# Autodesk Inventor assembly: robot_frame_layer2
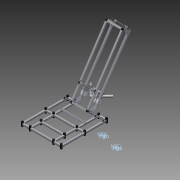
[picture p0: Inventor's stored thumbnail of the model, 180x180]
Saved by Autodesk Inventor 2011 (Build 150239000, 239)
## iProperties
Created: 2013-01-17
Part Number: robot_frame_layer2
Document SubType Name: Assembly
Designer: Christopher
Author: Christopher
## Documents named in this file (19)
- F:\Users\Christopher\Documents\GitHub\2013CAD\2013 robot\forklift\robot parts\robot_frame_layer2.iam
- F:\Users\Christopher\Documents\GitHub\2013CAD\2013 robot\forklift\robot parts\1tube_4_layer1_outside.ipt
- F:\Users\Christopher\Documents\GitHub\2013CAD\2013 robot\forklift\robot parts\1tube_6_layer1_boardsupportsupport.ipt
- F:\Users\Christopher\Documents\GitHub\2013CAD\2013 robot\forklift\robot parts\1tube_6_layer1_motorsupport.ipt
- F:\Users\Christopher\Documents\GitHub\2013CAD\2013 robot\forklift\robot parts\1tube_14_layer1_innersupport.ipt
- F:\Users\Christopher\Documents\GitHub\2013CAD\2013 robot\forklift\robot parts\1tube_14_layer1_inside.ipt
- F:\Users\Christopher\Documents\GitHub\2013CAD\2013 robot\forklift\robot parts\1tube_14_layer1_outside.ipt
- F:\Users\Christopher\Documents\GitHub\2013CAD\2013 robot\forklift\Misc parts\4-way corner.ipt
- F:\Users\Christopher\Documents\GitHub\2013CAD\2013 robot\forklift\Misc parts\5-way corner.ipt
- F:\Users\Christopher\Documents\GitHub\2013CAD\2013 robot\forklift\Misc parts\.5inch_side_bearing.ipt
- F:\Users\Christopher\Documents\GitHub\2013CAD\2013 robot\forklift\Misc parts\1.5_bolt_.25_20.ipt
- F:\Users\Christopher\Documents\GitHub\2013CAD\2013 robot\forklift\Misc parts\nut_.25_20.ipt
- F:\Users\Christopher\Documents\GitHub\2013CAD\2013 robot\forklift\Misc parts\.5_inch_axle_bushing.ipt
- F:\Users\Christopher\Documents\GitHub\2013CAD\2013 robot\forklift\robot parts\1tube_13_layer2_side.ipt
- F:\Users\Christopher\Documents\GitHub\2013CAD\2013 robot\forklift\Misc parts\6-way corner.ipt
- F:\Users\Christopher\Documents\GitHub\2013CAD\2013 robot\forklift\frame parts\0.5unkeyedaxle_26.ipt
- F:\Users\Christopher\Documents\GitHub\2013CAD\2013 robot\forklift\frame parts\forklift_1_0.iam
- F:\Users\Christopher\Documents\GitHub\2013CAD\2013 robot\forklift\Misc parts\steel_p60_mounting _plate.ipt
- F:\Users\Christopher\Documents\GitHub\2013CAD\2013 robot\forklift\Misc parts\hack_p60.ipt
## Components (66 placed, 18 different names)
1. 1tube_4_layer1_outside:1 — Mate:231, Mate:232, Mate:233, Mate:237, Mate:238, Mate:239
2. 1tube_6_layer1_boardsupportsupport:1 — Mate:225, Mate:226, Mate:227
3. 1tube_6_layer1_motorsupport:1 — Mate:221, Mate:222, Mate:223
4. 1tube_14_layer1_innersupport:1 — Mate:182, Mate:186, Mate:195, Mate:218, Mate:219, Mate:224
5. 1tube_14_layer1_outside:1 — Mate:234, Mate:235, Mate:236
6. 1tube_4_layer1_outside:2 — Mate:204, Flush:20, Mate:205, Mate:206, Mate:207, Mate:208
7. 1tube_14_layer1_innersupport:2 — Mate:175, Mate:176, Mate:185, Mate:192, Mate:193, Mate:194
8. 1tube_6_layer1_motorsupport:2 — Mate:173, Mate:177, Mate:179, Mate:183, Flush:17, Mate:184
9. 1tube_6_layer1_boardsupportsupport:2 — Mate:187, Mate:188, Mate:189, Mate:190, Mate:191
10. 1tube_4_layer1_outside:3 — Mate:164, Mate:165, Mate:166, Flush:18
11. 1tube_4_layer1_outside:4 — Mate:149, Mate:150, Mate:151, Mate:155, Mate:156, Flush:12
12. 1tube_4_layer1_outside:5 — Mate:159, Mate:160, Mate:161, Mate:178, Mate:241
13. 1tube_4_layer1_outside:6 — Mate:196, Mate:197, Mate:198, Mate:199, Mate:200, Mate:201, Mate:202
14. 1tube_14_layer1_inside:2 — Mate:162, Mate:167, Flush:16, Mate:168, Mate:169, Mate:170, Mate:171
15. 1tube_14_layer1_inside:3 — Flush:19, Mate:203, Mate:220, Mate:228, Mate:229, Mate:230
16. .5inch_side_bearing:1 — Insert:5, Insert:6, Insert:18, Insert:41, Insert:42, Insert:59
17. .5inch_side_bearing:2 — Insert:7, Insert:8, Insert:19, Insert:36, Insert:45, Insert:46
18. 1.5_bolt_.25_20:1 — Insert:6
19. 1.5_bolt_.25_20:2 — Insert:5
20. 1.5_bolt_.25_20:3 — Insert:7
21. 1.5_bolt_.25_20:4 — Insert:8
22. .5_inch_axle_bushing:1 — Insert:18
23. .5_inch_axle_bushing:2 — Insert:19
24. .5_inch_axle_bushing:6 — Insert:57, Insert:58, Insert:59
25. .5inch_side_bearing:3 — Insert:27, Insert:28, Insert:37, Insert:39, Insert:43, Insert:44
26. .5inch_side_bearing:4 — Insert:29, Insert:30, Insert:38, Insert:40, Insert:47, Insert:48
27. 1.5_bolt_.25_20:5 — Insert:28
28. 1.5_bolt_.25_20:6 — Insert:30
29. 1.5_bolt_.25_20:7 — Insert:29
30. 1.5_bolt_.25_20:8 — Insert:27
31. nut_.25_20:8 — Insert:56
32. .5_inch_axle_bushing:7 — Insert:36
33. .5_inch_axle_bushing:8 — Insert:37
34. .5_inch_axle_bushing:9 — Insert:38
35. .5_inch_axle_bushing:10 — Insert:39
36. .5_inch_axle_bushing:11 — Insert:40
37. 5-way corner:3 — Mate:218, Mate:219, Mate:224, Mate:225, Mate:226, Mate:227
38. 4-way corner:10 — Mate:155, Mate:156, Flush:12, Mate:157, Mate:158, Flush:13
39. 4-way corner:11 — Mate:149, Mate:150, Mate:151, Mate:152, Mate:153, Mate:154
40. 1tube_13_layer2_side:1 — Mate:157, Mate:158, Flush:13, Mate:172, Mate:174, Insert:43, Insert:44, Insert:49, Insert:50, Mate:240, Flush:21
41. 1tube_13_layer2_side:2 — Mate:152, Mate:153, Mate:154, Mate:163, Flush:14, Flush:15, Insert:41, Insert:42, Insert:51, Insert:52
42. 1tube_13_layer2_side:3 — Mate:212, Mate:213, Mate:214, Insert:47, Insert:48, Insert:55, Insert:56
43. 1tube_13_layer2_side:4 — Mate:209, Mate:210, Mate:211, Mate:215, Mate:216, Mate:217, Insert:45, Insert:46, Insert:53, Insert:54
44. 5-way corner:4 — Mate:159, Mate:160, Mate:161, Mate:162, Mate:163, Flush:14, Flush:15, Mate:168, Mate:169, Mate:170
45. 4-way corner:12 — Mate:164, Mate:165, Mate:166, Mate:167, Flush:16, Mate:171
46. 6-way corner:1 — Mate:172, Mate:173, Mate:174, Mate:175, Mate:176, Mate:177, Mate:178, Mate:179, Mate:185
47. 5-way corner:5 — Mate:182, Mate:183, Flush:17, Mate:184, Mate:186, Mate:187, Mate:188, Mate:189, Mate:195
48. 5-way corner:6 — Mate:190, Mate:191, Flush:18, Mate:234, Mate:235, Mate:236
49. 6-way corner:2 — Mate:192, Mate:193, Mate:194, Mate:196, Mate:197, Mate:198, Mate:215, Mate:216, Mate:217, Mate:221, Mate:222, Mate:223
50. 5-way corner:7 — Mate:199, Flush:19, Mate:200, Mate:201, Mate:202, Mate:203, Mate:220
51. 4-way corner:13 — Mate:204, Flush:20, Mate:205, Mate:209, Mate:210, Mate:211
52. 4-way corner:14 — Mate:206, Mate:207, Mate:208, Mate:212, Mate:213, Mate:214
53. 4-way corner:15 — Mate:228, Mate:229, Mate:230, Mate:231, Mate:232, Mate:233
54. 5-way corner:8 — Mate:237, Mate:238, Mate:239
55. nut_.25_20:9 — Insert:49
56. nut_.25_20:10 — Insert:50
57. nut_.25_20:11 — Insert:51
58. nut_.25_20:12 — Insert:52
59. nut_.25_20:13 — Insert:53
60. nut_.25_20:14 — Insert:55
61. nut_.25_20:15 — Insert:54
62. 0.5unkeyedaxle_26:1 — Insert:57
63. forklift_1_0:1 [sub-assembly] — Insert:58
64. steel_p60_mounting _plate:1 — Mate:240, Flush:21, Mate:241, Mate:242, Flush:22, Flush:23, Mate:243, Flush:24, Flush:25
65. hack_p60:1 — Mate:242, Flush:22, Flush:23
66. hack_p60:2 — Mate:243, Flush:24, Flush:25
## Relationships (141: Mate 93, Insert 34, Flush 14)
- Insert:5: .5inch_side_bearing:1 ↔ 1.5_bolt_.25_20:2
- Insert:6: .5inch_side_bearing:1 ↔ 1.5_bolt_.25_20:1
- Insert:7: .5inch_side_bearing:2 ↔ 1.5_bolt_.25_20:3
- Insert:8: .5inch_side_bearing:2 ↔ 1.5_bolt_.25_20:4
- Insert:18: .5inch_side_bearing:1 ↔ .5_inch_axle_bushing:1
- Insert:19: .5inch_side_bearing:2 ↔ .5_inch_axle_bushing:2
- Insert:27: .5inch_side_bearing:3 ↔ 1.5_bolt_.25_20:8
- Insert:28: .5inch_side_bearing:3 ↔ 1.5_bolt_.25_20:5
- Insert:29: .5inch_side_bearing:4 ↔ 1.5_bolt_.25_20:7
- Insert:30: .5inch_side_bearing:4 ↔ 1.5_bolt_.25_20:6
- Insert:36: .5inch_side_bearing:2 ↔ .5_inch_axle_bushing:7
- Insert:37: .5inch_side_bearing:3 ↔ .5_inch_axle_bushing:8
- Insert:38: .5inch_side_bearing:4 ↔ .5_inch_axle_bushing:9
- Insert:39: .5inch_side_bearing:3 ↔ .5_inch_axle_bushing:10
- Insert:40: .5inch_side_bearing:4 ↔ .5_inch_axle_bushing:11
- Mate:149: 1tube_4_layer1_outside:4 ↔ 4-way corner:11
- Mate:150: 1tube_4_layer1_outside:4 ↔ 4-way corner:11
- Mate:151: 1tube_4_layer1_outside:4 ↔ 4-way corner:11
- Mate:152: 4-way corner:11 ↔ 1tube_13_layer2_side:2
- Mate:153: 4-way corner:11 ↔ 1tube_13_layer2_side:2
- Mate:154: 4-way corner:11 ↔ 1tube_13_layer2_side:2
- Mate:155: 1tube_4_layer1_outside:4 ↔ 4-way corner:10
- Mate:156: 1tube_4_layer1_outside:4 ↔ 4-way corner:10
- Flush:12: 1tube_4_layer1_outside:4 ↔ 4-way corner:10
- Mate:157: 4-way corner:10 ↔ 1tube_13_layer2_side:1
- Mate:158: 4-way corner:10 ↔ 1tube_13_layer2_side:1
- Flush:13: 4-way corner:10 ↔ 1tube_13_layer2_side:1
- Mate:159: 1tube_4_layer1_outside:5 ↔ 5-way corner:4
- Mate:160: 1tube_4_layer1_outside:5 ↔ 5-way corner:4
- Mate:161: 1tube_4_layer1_outside:5 ↔ 5-way corner:4
- Mate:162: 1tube_14_layer1_inside:2 ↔ 5-way corner:4
- Mate:163: 1tube_13_layer2_side:2 ↔ 5-way corner:4
- Flush:14: 1tube_13_layer2_side:2 ↔ 5-way corner:4
- Flush:15: 1tube_13_layer2_side:2 ↔ 5-way corner:4
- Mate:164: 1tube_4_layer1_outside:3 ↔ 4-way corner:12
- Mate:165: 1tube_4_layer1_outside:3 ↔ 4-way corner:12
- Mate:166: 1tube_4_layer1_outside:3 ↔ 4-way corner:12
- Mate:167: 1tube_14_layer1_inside:2 ↔ 4-way corner:12
- Flush:16: 1tube_14_layer1_inside:2 ↔ 4-way corner:12
- Mate:168: 1tube_14_layer1_inside:2 ↔ 5-way corner:4
- Mate:169: 1tube_14_layer1_inside:2 ↔ 5-way corner:4
- Mate:170: 1tube_14_layer1_inside:2 ↔ 5-way corner:4
- Mate:171: 1tube_14_layer1_inside:2 ↔ 4-way corner:12
- Mate:172: 1tube_13_layer2_side:1 ↔ 6-way corner:1
- Mate:173: 1tube_6_layer1_motorsupport:2 ↔ 6-way corner:1
- Mate:174: 1tube_13_layer2_side:1 ↔ 6-way corner:1
- Mate:175: 1tube_14_layer1_innersupport:2 ↔ 6-way corner:1
- Mate:176: 1tube_14_layer1_innersupport:2 ↔ 6-way corner:1
- Mate:177: 1tube_6_layer1_motorsupport:2 ↔ 6-way corner:1
- Mate:178: 1tube_4_layer1_outside:5 ↔ 6-way corner:1
- Mate:179: 1tube_6_layer1_motorsupport:2 ↔ 6-way corner:1
- Mate:182: 1tube_14_layer1_innersupport:1 ↔ 5-way corner:5
- Mate:183: 1tube_6_layer1_motorsupport:2 ↔ 5-way corner:5
- Flush:17: 1tube_6_layer1_motorsupport:2 ↔ 5-way corner:5
- Mate:184: 1tube_6_layer1_motorsupport:2 ↔ 5-way corner:5
- Mate:185: 1tube_14_layer1_innersupport:2 ↔ 6-way corner:1
- Mate:186: 1tube_14_layer1_innersupport:1 ↔ 5-way corner:5
- Mate:187: 1tube_6_layer1_boardsupportsupport:2 ↔ 5-way corner:5
- Mate:188: 1tube_6_layer1_boardsupportsupport:2 ↔ 5-way corner:5
- Mate:189: 1tube_6_layer1_boardsupportsupport:2 ↔ 5-way corner:5
- Mate:190: 1tube_6_layer1_boardsupportsupport:2 ↔ 5-way corner:6
- Mate:191: 1tube_6_layer1_boardsupportsupport:2 ↔ 5-way corner:6
- Flush:18: 1tube_4_layer1_outside:3 ↔ 5-way corner:6
- Mate:192: 1tube_14_layer1_innersupport:2 ↔ 6-way corner:2
- Mate:193: 1tube_14_layer1_innersupport:2 ↔ 6-way corner:2
- Mate:194: 1tube_14_layer1_innersupport:2 ↔ 6-way corner:2
- Mate:195: 1tube_14_layer1_innersupport:1 ↔ 5-way corner:5
- Mate:196: 1tube_4_layer1_outside:6 ↔ 6-way corner:2
- Mate:197: 1tube_4_layer1_outside:6 ↔ 6-way corner:2
- Mate:198: 1tube_4_layer1_outside:6 ↔ 6-way corner:2
- Mate:199: 1tube_4_layer1_outside:6 ↔ 5-way corner:7
- Flush:19: 1tube_14_layer1_inside:3 ↔ 5-way corner:7
- Mate:200: 1tube_4_layer1_outside:6 ↔ 5-way corner:7
- Mate:201: 1tube_4_layer1_outside:6 ↔ 5-way corner:7
- Mate:202: 1tube_4_layer1_outside:6 ↔ 5-way corner:7
- Mate:203: 1tube_14_layer1_inside:3 ↔ 5-way corner:7
- Mate:204: 1tube_4_layer1_outside:2 ↔ 4-way corner:13
- Flush:20: 1tube_4_layer1_outside:2 ↔ 4-way corner:13
- Mate:205: 1tube_4_layer1_outside:2 ↔ 4-way corner:13
- Mate:206: 1tube_4_layer1_outside:2 ↔ 4-way corner:14
- Mate:207: 1tube_4_layer1_outside:2 ↔ 4-way corner:14
- Mate:208: 1tube_4_layer1_outside:2 ↔ 4-way corner:14
- Mate:209: 1tube_13_layer2_side:4 ↔ 4-way corner:13
- Mate:210: 1tube_13_layer2_side:4 ↔ 4-way corner:13
- Mate:211: 1tube_13_layer2_side:4 ↔ 4-way corner:13
- Mate:212: 1tube_13_layer2_side:3 ↔ 4-way corner:14
- Mate:213: 1tube_13_layer2_side:3 ↔ 4-way corner:14
- Mate:214: 1tube_13_layer2_side:3 ↔ 4-way corner:14
- Mate:215: 1tube_13_layer2_side:4 ↔ 6-way corner:2
- Mate:216: 1tube_13_layer2_side:4 ↔ 6-way corner:2
- Mate:217: 1tube_13_layer2_side:4 ↔ 6-way corner:2
- Mate:218: 1tube_14_layer1_innersupport:1 ↔ 5-way corner:3
- Mate:219: 1tube_14_layer1_innersupport:1 ↔ 5-way corner:3
- Mate:220: 1tube_14_layer1_inside:3 ↔ 5-way corner:7
- Mate:221: 1tube_6_layer1_motorsupport:1 ↔ 6-way corner:2
- Mate:222: 1tube_6_layer1_motorsupport:1 ↔ 6-way corner:2
- Mate:223: 1tube_6_layer1_motorsupport:1 ↔ 6-way corner:2
- Mate:224: 1tube_14_layer1_innersupport:1 ↔ 5-way corner:3
- Mate:225: 1tube_6_layer1_boardsupportsupport:1 ↔ 5-way corner:3
- Mate:226: 1tube_6_layer1_boardsupportsupport:1 ↔ 5-way corner:3
- Mate:227: 1tube_6_layer1_boardsupportsupport:1 ↔ 5-way corner:3
- Mate:228: 1tube_14_layer1_inside:3 ↔ 4-way corner:15
- Mate:229: 1tube_14_layer1_inside:3 ↔ 4-way corner:15
- Mate:230: 1tube_14_layer1_inside:3 ↔ 4-way corner:15
- Mate:231: 1tube_4_layer1_outside:1 ↔ 4-way corner:15
- Mate:232: 1tube_4_layer1_outside:1 ↔ 4-way corner:15
- Mate:233: 1tube_4_layer1_outside:1 ↔ 4-way corner:15
- Mate:234: 1tube_14_layer1_outside:1 ↔ 5-way corner:6
- Mate:235: 1tube_14_layer1_outside:1 ↔ 5-way corner:6
- Mate:236: 1tube_14_layer1_outside:1 ↔ 5-way corner:6
- Mate:237: 1tube_4_layer1_outside:1 ↔ 5-way corner:8
- Mate:238: 1tube_4_layer1_outside:1 ↔ 5-way corner:8
- Mate:239: 1tube_4_layer1_outside:1 ↔ 5-way corner:8
- Insert:41: .5inch_side_bearing:1 ↔ 1tube_13_layer2_side:2
- Insert:42: .5inch_side_bearing:1 ↔ 1tube_13_layer2_side:2
- Insert:43: .5inch_side_bearing:3 ↔ 1tube_13_layer2_side:1
- Insert:44: .5inch_side_bearing:3 ↔ 1tube_13_layer2_side:1
- Insert:45: .5inch_side_bearing:2 ↔ 1tube_13_layer2_side:4
- Insert:46: .5inch_side_bearing:2 ↔ 1tube_13_layer2_side:4
- Insert:47: .5inch_side_bearing:4 ↔ 1tube_13_layer2_side:3
- Insert:48: .5inch_side_bearing:4 ↔ 1tube_13_layer2_side:3
- Insert:49: 1tube_13_layer2_side:1 ↔ nut_.25_20:9
- Insert:50: 1tube_13_layer2_side:1 ↔ nut_.25_20:10
- Insert:51: 1tube_13_layer2_side:2 ↔ nut_.25_20:11
- Insert:52: 1tube_13_layer2_side:2 ↔ nut_.25_20:12
- Insert:53: 1tube_13_layer2_side:4 ↔ nut_.25_20:13
- Insert:54: 1tube_13_layer2_side:4 ↔ nut_.25_20:15
- Insert:55: 1tube_13_layer2_side:3 ↔ nut_.25_20:14
- Insert:56: nut_.25_20:8 ↔ 1tube_13_layer2_side:3
- Insert:57: .5_inch_axle_bushing:6 ↔ 0.5unkeyedaxle_26:1
- Insert:58 (190.5 mm): .5_inch_axle_bushing:6 ↔ forklift_1_0:1
- Mate:240: 1tube_13_layer2_side:1 ↔ steel_p60_mounting _plate:1
- Flush:21: 1tube_13_layer2_side:1 ↔ steel_p60_mounting _plate:1
- Mate:241 (101.6 mm): 1tube_4_layer1_outside:5 ↔ steel_p60_mounting _plate:1
- Mate:242: steel_p60_mounting _plate:1 ↔ hack_p60:1
- Flush:22: steel_p60_mounting _plate:1 ↔ hack_p60:1
- Flush:23: steel_p60_mounting _plate:1 ↔ hack_p60:1
- Mate:243: steel_p60_mounting _plate:1 ↔ hack_p60:2
- Flush:24: steel_p60_mounting _plate:1 ↔ hack_p60:2
- Flush:25: steel_p60_mounting _plate:1 ↔ hack_p60:2
- Insert:59: .5inch_side_bearing:1 ↔ .5_inch_axle_bushing:6
